# Autodesk Inventor assembly: Gimbal Assembly
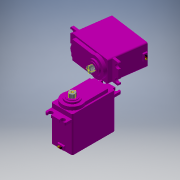
[picture p0: Inventor's stored thumbnail of the model, 180x180]
Saved by Autodesk Inventor 2016 (Build 200138000, 138)
## iProperties
Created: 2016-02-11
Part Number: Gimbal Assembly
Document SubType Name: Assembly
Designer: RoksBot
Author: RoksBot
## Documents named in this file (3)
- C:\Users\RoksBot\Documents\Inventor\Camera Mount\Gimbal Assembly.iam
- C:\Users\RoksBot\Documents\Inventor\Camera Mount\Servo Horn.ipt
- C:\Users\RoksBot\Documents\Inventor\Camera Mount\servo.ipt
## Components (4 placed, 2 different names)
1. Servo Horn:1 — Insert:2
2. servo:1 — Insert:1, Mate:1
3. Servo Horn:2 — Insert:1, Flush:1, Mate:2
4. servo:2 — Insert:2, Mate:1, Flush:1, Mate:2
## Relationships (5: Insert 2, Mate 2, Flush 1)
- Insert:1: servo:1 ↔ Servo Horn:2
- Insert:2: Servo Horn:1 ↔ servo:2
- Mate:1 (7.62 mm): servo:1 ↔ servo:2
- Flush:1 (-9.7282 mm): Servo Horn:2 ↔ servo:2
- Mate:2 (19.05 mm): Servo Horn:2 ↔ servo:2
